# Autodesk Inventor assembly: ЛЦМК.30000.10.00.01 Згт под основание
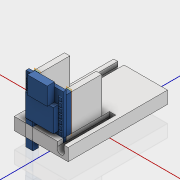
[picture p0: Inventor's stored thumbnail of the model, 180x180]
Saved by Autodesk Inventor 2021.2 (Build 252289000, 289)
## iProperties
Created: 2025-11-22
Part Number: ЛЦМК.30000.10.00.01 Згт под основание
Document SubType Name: Assembly
Designer: Захаров
Author: Захаров
## Documents named in this file (3)
- C:\Users\User\Documents\CaseARHead1\Заготовки\ЛЦМК.30000.10.00.01 Згт под основание.iam
- C:\Users\User\Documents\CaseARHead1\Заготовки\Згт xiao под основание.iam
- C:\Users\User\Documents\CaseARHead1\Заготовки\ЛЦМК.30000.10.00.01 Згт по одснование.ipt
## Components (2 placed, 2 different names)
1. Згт xiao под основание:1 [sub-assembly] — Заподлицо:1, Заподлицо:2, Совмещение:1
2. ЛЦМК.30000.10.00.01 Згт по одснование:1 — Заподлицо:1, Заподлицо:2, Совмещение:1
## Relationships (3: Flush 2, Mate 1)
- Заподлицо:1 [Flush]: Згт xiao под основание:1 ↔ ЛЦМК.30000.10.00.01 Згт по одснование:1
- Заподлицо:2 [Flush] (3 mm): Згт xiao под основание:1 ↔ ЛЦМК.30000.10.00.01 Згт по одснование:1
- Совмещение:1 [Mate] (-2 mm): Згт xiao под основание:1 ↔ ЛЦМК.30000.10.00.01 Згт по одснование:1
